# Autodesk Inventor assembly: DRC2020
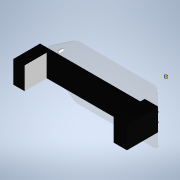
[picture p0: Inventor's stored thumbnail of the model, 180x180]
Saved by Autodesk Inventor 2020 (Build 240168000, 168)
## iProperties
Created: 2019-08-05
Part Number: DRC2020
Document SubType Name: Assembly
Designer: n10208577
Author: n10208577
## Documents named in this file (4)
- C:\Users\n10208577\Desktop\DRC\DRC2020-Hardware\Design\DRC2020.iam
- C:\Users\n10208577\Desktop\DRC\DRC2020-Hardware\Design\base.ipt
- C:\Users\n10208577\Desktop\DRC\DRC2020-Hardware\Design\10mmStandOff.ipt
- C:\Users\n10208577\Desktop\DRC\DRC2020-Hardware\Design\carSpacer.ipt
## Components (6 placed, 3 different names)
1. base:1 — Insert:1, Insert:2, Insert:3, Insert:4, Insert:5, Insert:6
2. 10mmStandOff:1 — Insert:2
3. 10mmStandOff:2 — Insert:1
4. 10mmStandOff:3 — Insert:4
5. 10mmStandOff:4 — Insert:3
6. carSpacer:1 — Insert:5, Insert:6
## Relationships (6: Insert 6)
- Insert:1: base:1 ↔ 10mmStandOff:2
- Insert:2: base:1 ↔ 10mmStandOff:1
- Insert:3: base:1 ↔ 10mmStandOff:4
- Insert:4: base:1 ↔ 10mmStandOff:3
- Insert:5: base:1 ↔ carSpacer:1
- Insert:6: base:1 ↔ carSpacer:1
